# Autodesk Inventor assembly: AdaptadorBancoDePruebas
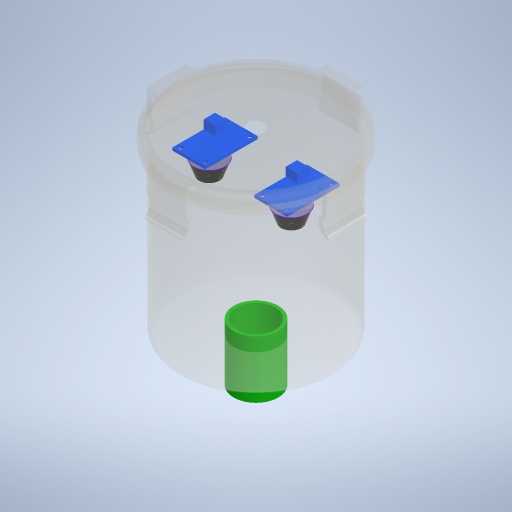
[picture p0: Inventor's stored thumbnail of the model, 512x512]
Saved by Autodesk Inventor 2024 (Build 280153000, 153)
## iProperties
Created: 2024-05-15
Part Number: AdaptadorBancoDePruebas
Document SubType Name: Assembly
Designer: alexa
Author: alexa
## Documents named in this file (5)
- C:\Users\alexa\OneDrive\Escritorio\Biogas\AdaptadorBancoDePruebas.iam
- C:\Users\alexa\OneDrive\Escritorio\Biogas\ContenedorTest.ipt
- C:\Users\alexa\OneDrive\Escritorio\Biogas\TapaContenedorTest.ipt
- C:\Users\alexa\OneDrive\Escritorio\Biogas\ConectorGasCamara.ipt
- C:\Users\alexa\OneDrive\Escritorio\Biogas\SensorGas.ipt
## Components (5 placed, 4 different names)
1. ContenedorTest:1 — Mate:1, Mate:2, Mate:3, Mate:4
2. TapaContenedorTest:1 — Mate:2, Mate:3, Mate:5, Mate:6, Mate:9
3. ConectorGasCamara:1 — Mate:4
4. SensorGas:1 — Mate:5, Mate:7, Flush:1
5. SensorGas:2 — Mate:6, Flush:2, Flush:3, Flush:4, Mate:8
## Relationships (13: Mate 9, Flush 4)
- Mate:1: ContenedorTest:1
- Mate:2: ContenedorTest:1 ↔ TapaContenedorTest:1
- Mate:3: ContenedorTest:1 ↔ TapaContenedorTest:1
- Mate:4: ContenedorTest:1 ↔ ConectorGasCamara:1
- Mate:5 (20 mm): TapaContenedorTest:1 ↔ SensorGas:1
- Mate:6 (20 mm): TapaContenedorTest:1 ↔ SensorGas:2
- Mate:7 (25 mm): SensorGas:1
- Flush:1: SensorGas:1
- Flush:2: SensorGas:2
- Flush:3: SensorGas:2
- Flush:4: SensorGas:2
- Mate:8 (-25 mm): SensorGas:2
- Mate:9: TapaContenedorTest:1
